# Autodesk Inventor assembly: SliddingAssembly
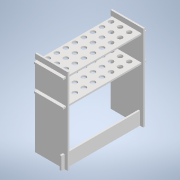
[picture p0: Inventor's stored thumbnail of the model, 180x180]
Saved by Autodesk Inventor 2020 (Build 240168000, 168)
## iProperties
Created: 2019-08-12
Part Number: SliddingAssembly
Document SubType Name: Assembly
Designer: eugen
Author: eugen
## Documents named in this file (4)
- \\udrive.uw.edu\udrive\IMACRack\FinalDesign\FinalAssembly.iam
- \\udrive.uw.edu\udrive\IMACRack\FinalDesign\BackBrace.ipt
- \\udrive.uw.edu\udrive\IMACRack\FinalDesign\Rack.ipt
- \\udrive.uw.edu\udrive\IMACRack\FinalDesign\Sides.ipt
## Components (5 placed, 3 different names)
1. Rack:1 — Mate:15, Mate:16, Mate:17
2. Sides:1 — Mate:11, Mate:12, Mate:13
3. Rack:2 — Mate:18, Mate:19, Mate:20
4. Sides:2 — Mate:10, Mate:14, Mate:15, Mate:16, Mate:17, Mate:18, Mate:19, Mate:20, Mate:21
5. BackBrace:1 — Mate:10, Mate:11, Mate:12, Mate:13, Mate:14, Mate:21
## Relationships (12: Mate 12)
- Mate:10: Sides:2 ↔ BackBrace:1
- Mate:11: Sides:1 ↔ BackBrace:1
- Mate:12: Sides:1 ↔ BackBrace:1
- Mate:13: Sides:1 ↔ BackBrace:1
- Mate:14: Sides:2 ↔ BackBrace:1
- Mate:15: Rack:1 ↔ Sides:2
- Mate:16: Rack:1 ↔ Sides:2
- Mate:17: Rack:1 ↔ Sides:2
- Mate:18: Rack:2 ↔ Sides:2
- Mate:19: Rack:2 ↔ Sides:2
- Mate:20: Rack:2 ↔ Sides:2
- Mate:21: Sides:2 ↔ BackBrace:1
